# Autodesk Inventor assembly: Baugruppe1
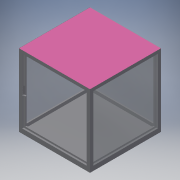
[picture p0: Inventor's stored thumbnail of the model, 180x180]
Saved by Autodesk Inventor 2018.3 (Build 223284000, 284)
## iProperties
Created: 2019-09-20
Part Number: Baugruppe1
Material: Generisch
Document SubType Name: Assembly
Designer: Lolob
Author: Lolob
Title: SmartCube
## Documents named in this file (11)
- D:\Dokumente\S ch u l e\Dipl\Smartcube_Construction\Version_3\Baugruppe1.iam
- D:\Dokumente\S ch u l e\Dipl\Smartcube_Construction\Version_2\PV_Modul_CPY_3.ipt
- D:\Dokumente\S ch u l e\Dipl\Smartcube_Construction\Version_3\Boden.ipt
- D:\Dokumente\S ch u l e\Dipl\Smartcube_Construction\Version_2\PV_Modul_CPY_3_CPY.ipt
- D:\Dokumente\S ch u l e\Dipl\Smartcube_Construction\Version_2\PV_Modul_CPY_3_CPY1.ipt
- D:\Dokumente\S ch u l e\Dipl\Smartcube_Construction\Version_2\PV_Modul_CPY_3_CPY2.ipt
- D:\Dokumente\S ch u l e\Dipl\Smartcube_Construction\Version_3\Boden_2.ipt
- D:\Dokumente\S ch u l e\Dipl\Smartcube_Construction\Version_3\PV_Rahmen.ipt
- D:\Dokumente\S ch u l e\Dipl\Smartcube_Construction\Version_3\PV_Rahmen_CPY.ipt
- D:\Dokumente\S ch u l e\Dipl\Smartcube_Construction\Version_3\PV_Rahmen_CPY1.ipt
- D:\Dokumente\S ch u l e\Dipl\Smartcube_Construction\Version_3\PV_Rahmen_CPY2.ipt
## Components (10 placed, 10 different names)
1. Sitzfläche:1 — Starr:9
2. PV_Modul_CPY_3:1 — Starr:1
3. PV_Modul_CPY_3_CPY:1 — Starr:5
4. PV_Modul_CPY_3_CPY1:1 — Starr:7
5. PV_Modul_CPY_3_CPY2:1 — Starr:6
6. Boden_2:1 — Starr:8
7. PV_Rahmen:1 — Starr:1, Starr:2
8. PV_Rahmen_CPY:1 — Starr:2, Starr:3, Starr:7, Starr:8, Starr:9
9. PV_Rahmen_CPY1:1 — Starr:3, Starr:4, Starr:6
10. PV_Rahmen_CPY2:1 — Starr:4, Starr:5
## Relationships (9: WeldJoint 9)
- Starr:1 [WeldJoint]: PV_Modul_CPY_3:1 ↔ PV_Rahmen:1
- Starr:2 [WeldJoint]: PV_Rahmen:1 ↔ PV_Rahmen_CPY:1
- Starr:3 [WeldJoint]: PV_Rahmen_CPY:1 ↔ PV_Rahmen_CPY1:1
- Starr:4 [WeldJoint]: PV_Rahmen_CPY1:1 ↔ PV_Rahmen_CPY2:1
- Starr:5 [WeldJoint]: PV_Modul_CPY_3_CPY:1 ↔ PV_Rahmen_CPY2:1
- Starr:6 [WeldJoint]: PV_Modul_CPY_3_CPY2:1 ↔ PV_Rahmen_CPY1:1
- Starr:7 [WeldJoint]: PV_Modul_CPY_3_CPY1:1 ↔ PV_Rahmen_CPY:1
- Starr:8 [WeldJoint]: Boden_2:1 ↔ PV_Rahmen_CPY:1
- Starr:9 [WeldJoint]: Sitzfläche:1 ↔ PV_Rahmen_CPY:1
